# Autodesk Inventor assembly: 2 x 15 custom!!!
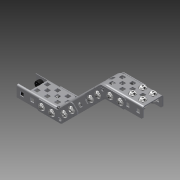
[picture p0: Inventor's stored thumbnail of the model, 180x180]
Saved by Autodesk Inventor 2012 (Build 160160000, 160)
## iProperties
Created: 2011-09-02
Part Number: 2 x 15 custom!!!
Document SubType Name: Assembly
Designer: Dakota.Bayer
Author: Dakota.Bayer
## Documents named in this file (5)
- C:\Users\Wade\Documents\1103 Robot - CAD Assembly\2 x 15 custom!!!.iam
- C:\Users\Wade\Documents\1103 Robot - CAD Assembly\2 x 15 bent 45 degrees.ipt
- C:\Users\Wade\Documents\24C VEX CAD Files\Metal Other\45 Degree Gusset.ipt
- C:\Users\Wade\Documents\1103 Robot - CAD Assembly\.375'' Screw & Nylock Nut.iam
- C:\Users\Wade\Documents\24C VEX CAD Files\Washers & Spacers\Spacer (Thin), 4.6mm.ipt
## Components (27 placed, 4 different names)
1. 2 x 15 bent 45 degrees:1 — Mate:2, Flush:1, Flush:2, Mate:3, Flush:3, Mate:4, Flush:5, Mate:5, Mate:38, Mate:39, Mate:41, Mate:42, Mate:44, Mate:45, Mate:47, Mate:48, Mate:50, Mate:53, Flush:6, Flush:7, Flush:8, Flush:9, Mate:55, Mate:56, Mate:57, Mate:58, Mate:59, Mate:60
2. 45 Degree Gusset:1 — Mate:2, Flush:1, Flush:2, Mate:30, Mate:31, Mate:32, Mate:33, Mate:34, Mate:35, Mate:36, Mate:37
3. 45 Degree Gusset:2 — Mate:3, Flush:3, Mate:22, Mate:23, Mate:24, Mate:25, Mate:26, Mate:27, Mate:28, Mate:29, Flush:8
4. 45 Degree Gusset:3 — Mate:4, Flush:5, Mate:6, Mate:7, Mate:8, Mate:9, Mate:10, Mate:11, Mate:12, Mate:13, Flush:9
5. 45 Degree Gusset:4 — Mate:5, Mate:14, Mate:15, Mate:16, Mate:17, Mate:18, Mate:19, Mate:20, Mate:21, Flush:6, Flush:7
6. .375'' Screw & Nylock Nut:1 [sub-assembly] — Mate:22, Mate:23
7. .375'' Screw & Nylock Nut:2 [sub-assembly] — Mate:26, Mate:27
8. .375'' Screw & Nylock Nut:3 [sub-assembly] — Mate:28, Mate:29
9. .375'' Screw & Nylock Nut:4 [sub-assembly] — Mate:24, Mate:25
10. .375'' Screw & Nylock Nut:5 [sub-assembly] — Mate:36, Mate:37
11. .375'' Screw & Nylock Nut:6 [sub-assembly] — Mate:34, Mate:35
12. .375'' Screw & Nylock Nut:7 [sub-assembly] — Mate:32, Mate:33
13. .375'' Screw & Nylock Nut:8 [sub-assembly] — Mate:30, Mate:31
14. .375'' Screw & Nylock Nut:9 [sub-assembly] — Mate:20, Mate:21
15. .375'' Screw & Nylock Nut:10 [sub-assembly] — Mate:18, Mate:19
16. .375'' Screw & Nylock Nut:11 [sub-assembly] — Mate:16, Mate:17
17. .375'' Screw & Nylock Nut:12 [sub-assembly] — Mate:14, Mate:15
18. .375'' Screw & Nylock Nut:13 [sub-assembly] — Mate:6, Mate:7
19. .375'' Screw & Nylock Nut:14 [sub-assembly] — Mate:8, Mate:9
20. .375'' Screw & Nylock Nut:15 [sub-assembly] — Mate:10, Mate:11
21. .375'' Screw & Nylock Nut:16 [sub-assembly] — Mate:12, Mate:13
22. .375'' Screw & Nylock Nut:17 [sub-assembly] — Mate:47, Mate:48, Mate:56
23. .375'' Screw & Nylock Nut:18 [sub-assembly] — Mate:44, Mate:45, Mate:58
24. .375'' Screw & Nylock Nut:19 [sub-assembly] — Mate:41, Mate:42, Mate:57
25. .375'' Screw & Nylock Nut:20 [sub-assembly] — Mate:38, Mate:39, Mate:55
26. Spacer (Thin), 4.6mm:1 — Mate:50, Mate:54
27. Spacer (Thin), 4.6mm:2 — Mate:53, Mate:54, Mate:59, Mate:60
## Relationships (61: Mate 53, Flush 8)
- Mate:2: 2 x 15 bent 45 degrees:1 ↔ 45 Degree Gusset:1
- Flush:1: 2 x 15 bent 45 degrees:1 ↔ 45 Degree Gusset:1
- Flush:2: 2 x 15 bent 45 degrees:1 ↔ 45 Degree Gusset:1
- Mate:3: 2 x 15 bent 45 degrees:1 ↔ 45 Degree Gusset:2
- Flush:3: 2 x 15 bent 45 degrees:1 ↔ 45 Degree Gusset:2
- Mate:4: 2 x 15 bent 45 degrees:1 ↔ 45 Degree Gusset:3
- Flush:5: 2 x 15 bent 45 degrees:1 ↔ 45 Degree Gusset:3
- Mate:5: 2 x 15 bent 45 degrees:1 ↔ 45 Degree Gusset:4
- Mate:6: 45 Degree Gusset:3 ↔ .375'' Screw & Nylock Nut:13
- Mate:7: 45 Degree Gusset:3 ↔ .375'' Screw & Nylock Nut:13
- Mate:8: 45 Degree Gusset:3 ↔ .375'' Screw & Nylock Nut:14
- Mate:9: 45 Degree Gusset:3 ↔ .375'' Screw & Nylock Nut:14
- Mate:10: 45 Degree Gusset:3 ↔ .375'' Screw & Nylock Nut:15
- Mate:11: 45 Degree Gusset:3 ↔ .375'' Screw & Nylock Nut:15
- Mate:12: 45 Degree Gusset:3 ↔ .375'' Screw & Nylock Nut:16
- Mate:13: 45 Degree Gusset:3 ↔ .375'' Screw & Nylock Nut:16
- Mate:14: 45 Degree Gusset:4 ↔ .375'' Screw & Nylock Nut:12
- Mate:15: 45 Degree Gusset:4 ↔ .375'' Screw & Nylock Nut:12
- Mate:16: 45 Degree Gusset:4 ↔ .375'' Screw & Nylock Nut:11
- Mate:17: 45 Degree Gusset:4 ↔ .375'' Screw & Nylock Nut:11
- Mate:18: 45 Degree Gusset:4 ↔ .375'' Screw & Nylock Nut:10
- Mate:19: 45 Degree Gusset:4 ↔ .375'' Screw & Nylock Nut:10
- Mate:20: 45 Degree Gusset:4 ↔ .375'' Screw & Nylock Nut:9
- Mate:21: 45 Degree Gusset:4 ↔ .375'' Screw & Nylock Nut:9
- Mate:22: 45 Degree Gusset:2 ↔ .375'' Screw & Nylock Nut:1
- Mate:23: 45 Degree Gusset:2 ↔ .375'' Screw & Nylock Nut:1
- Mate:24: 45 Degree Gusset:2 ↔ .375'' Screw & Nylock Nut:4
- Mate:25: 45 Degree Gusset:2 ↔ .375'' Screw & Nylock Nut:4
- Mate:26: 45 Degree Gusset:2 ↔ .375'' Screw & Nylock Nut:2
- Mate:27: 45 Degree Gusset:2 ↔ .375'' Screw & Nylock Nut:2
- Mate:28: 45 Degree Gusset:2 ↔ .375'' Screw & Nylock Nut:3
- Mate:29: 45 Degree Gusset:2 ↔ .375'' Screw & Nylock Nut:3
- Mate:30: 45 Degree Gusset:1 ↔ .375'' Screw & Nylock Nut:8
- Mate:31: 45 Degree Gusset:1 ↔ .375'' Screw & Nylock Nut:8
- Mate:32: 45 Degree Gusset:1 ↔ .375'' Screw & Nylock Nut:7
- Mate:33: 45 Degree Gusset:1 ↔ .375'' Screw & Nylock Nut:7
- Mate:34: 45 Degree Gusset:1 ↔ .375'' Screw & Nylock Nut:6
- Mate:35: 45 Degree Gusset:1 ↔ .375'' Screw & Nylock Nut:6
- Mate:36: 45 Degree Gusset:1 ↔ .375'' Screw & Nylock Nut:5
- Mate:37: 45 Degree Gusset:1 ↔ .375'' Screw & Nylock Nut:5
- Mate:38 (2.3114 mm): 2 x 15 bent 45 degrees:1 ↔ .375'' Screw & Nylock Nut:20
- Mate:39 (2.3114 mm): 2 x 15 bent 45 degrees:1 ↔ .375'' Screw & Nylock Nut:20
- Mate:41 (2.3114 mm): 2 x 15 bent 45 degrees:1 ↔ .375'' Screw & Nylock Nut:19
- Mate:42 (2.3114 mm): 2 x 15 bent 45 degrees:1 ↔ .375'' Screw & Nylock Nut:19
- Mate:44 (2.3114 mm): 2 x 15 bent 45 degrees:1 ↔ .375'' Screw & Nylock Nut:18
- Mate:45 (2.3114 mm): 2 x 15 bent 45 degrees:1 ↔ .375'' Screw & Nylock Nut:18
- Mate:47 (2.3114 mm): 2 x 15 bent 45 degrees:1 ↔ .375'' Screw & Nylock Nut:17
- Mate:48 (2.3114 mm): 2 x 15 bent 45 degrees:1 ↔ .375'' Screw & Nylock Nut:17
- Mate:50: 2 x 15 bent 45 degrees:1 ↔ Spacer (Thin), 4.6mm:1
- Mate:53: 2 x 15 bent 45 degrees:1 ↔ Spacer (Thin), 4.6mm:2
- Mate:54: Spacer (Thin), 4.6mm:1 ↔ Spacer (Thin), 4.6mm:2
- Flush:6: 2 x 15 bent 45 degrees:1 ↔ 45 Degree Gusset:4
- Flush:7: 2 x 15 bent 45 degrees:1 ↔ 45 Degree Gusset:4
- Flush:8: 2 x 15 bent 45 degrees:1 ↔ 45 Degree Gusset:2
- Flush:9: 2 x 15 bent 45 degrees:1 ↔ 45 Degree Gusset:3
- Mate:55 (1.1684 mm): 2 x 15 bent 45 degrees:1 ↔ .375'' Screw & Nylock Nut:20
- Mate:56 (1.1684 mm): 2 x 15 bent 45 degrees:1 ↔ .375'' Screw & Nylock Nut:17
- Mate:57 (1.1684 mm): 2 x 15 bent 45 degrees:1 ↔ .375'' Screw & Nylock Nut:19
- Mate:58 (1.1684 mm): 2 x 15 bent 45 degrees:1 ↔ .375'' Screw & Nylock Nut:18
- Mate:59 (2.3114 mm): 2 x 15 bent 45 degrees:1 ↔ Spacer (Thin), 4.6mm:2
- Mate:60 (2.3114 mm): 2 x 15 bent 45 degrees:1 ↔ Spacer (Thin), 4.6mm:2
